# Autodesk Inventor assembly: LowerBody_MIR
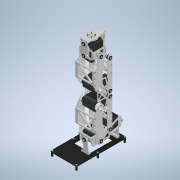
[picture p0: Inventor's stored thumbnail of the model, 180x180]
Saved by Autodesk Inventor 2020.4 (Build 244396000, 396)
## iProperties
Created: 2021-10-01
Part Number: LowerBody_MIR
Document SubType Name: Assembly
Designer: Masato
Mass: 1009.03 g
Surface Area: 2721.67 cm^2
Volume: 456.516 cm^3
Density: 2.21029 g/cm^3
Author: Masato
## Documents named in this file (14)
- C:\Users\Masato\Documents\Inventor\CIT Brains_Inventor\OpenPlatform_ver3_0\LowerBody\LowerBody_MIR.iam
- C:\Users\Masato\Documents\Inventor\CIT Brains_Inventor\OpenPlatform_ver3_0\LowerBody\Ankle\Ankle.iam
- C:\Users\Masato\Documents\Inventor\CIT Brains_Inventor\OpenPlatform_ver3_0\LowerBody\Ankle\Ankle_side_pitch.iam
- C:\Users\Masato\Documents\Inventor\CIT Brains_Inventor\OpenPlatform_ver3_0\LowerBody\Knee\Knee.iam
- C:\Users\Masato\Documents\Inventor\CIT Brains_Inventor\OpenPlatform_ver3_0\LowerBody\Leg_joit\Leg_joint_roll_pitch.iam
- C:\Users\Masato\Documents\Inventor\CIT Brains_Inventor\OpenPlatform_ver3_0\LowerBody\Leg_joit\Leg_joint_roll_yaw.iam
- C:\Users\Masato\Documents\Inventor\CIT Brains_Inventor\OpenPlatform_ver3_0\LowerBody\Slider_crank\Slider_crank_mechanism.iam
- C:\Users\Masato\Documents\Inventor\CIT Brains_Inventor\OpenPlatform_ver3_0\LowerBody\Link\BackLink.iam
- C:\Users\Masato\Documents\Inventor\CIT Brains_Inventor\OpenPlatform_ver3_0\LowerBody\Link\FrontLink.iam
- C:\Users\Masato\Documents\Inventor\CIT Brains_Inventor\OpenPlatform_ver3_0\Ready_Made\Screw\M2_6-6.ipt
- C:\Users\Masato\Documents\Inventor\CIT Brains_Inventor\OpenPlatform_ver3_0\Ready_Made\Screw\M3-6.ipt
- C:\Users\Masato\Documents\Inventor\CIT Brains_Inventor\OpenPlatform_ver3_0\Ready_Made\Screw\M2_6-10.ipt
- C:\Users\Masato\Documents\Inventor\CIT Brains_Inventor\OpenPlatform_ver3_0\Ready_Made\Screw\M3-8.ipt
- C:\Users\Masato\Documents\Inventor\CIT Brains_Inventor\OpenPlatform_ver3_0\LowerBody\Foot\Foot_MIR.iam
## Components (64 placed, 13 different names)
1. Ankle:1 [sub-assembly] — 挿入:21, 挿入:22, 挿入:67
2. Ankle_side_pitch:1 [sub-assembly] — 挿入:21, フラッシュ:5, 挿入:36, 挿入:35, 挿入:23, 挿入:24, 挿入:25, 挿入:26
3. Ankle_side_pitch:2 [sub-assembly] — フラッシュ:5, 挿入:22, 挿入:27, 挿入:28, 挿入:29, 挿入:30
4. Knee:1 [sub-assembly] — 挿入:33, 挿入:31, 挿入:34, 挿入:32
5. Leg_joint_roll_pitch:1 [sub-assembly] — 挿入:11, 挿入:2, 挿入:38, 挿入:37, 挿入:1
6. Leg_joint_roll_yaw:1 [sub-assembly] — 挿入:11, フラッシュ:4, フラッシュ:3, メイト:1, 角度:2, 挿入:12, 挿入:13, 挿入:14, 角度:8, 角度:9
7. Slider_crank_mechanism:1 [sub-assembly] — 挿入:2, 角度:1, 挿入:10, 挿入:9, 挿入:8, 挿入:7
8. BackLink:1 [sub-assembly] — 挿入:36, 挿入:33, 挿入:42, 挿入:46, 挿入:64, 挿入:66
9. FrontLink:1 [sub-assembly] — 挿入:35, 挿入:31, 挿入:51, 挿入:52, 挿入:53, 挿入:54, 挿入:59, 挿入:60, 挿入:61, 挿入:62, 挿入:63, 挿入:65, 角度:6
10. BackLink:2 [sub-assembly] — 挿入:38, 挿入:34, 挿入:39, 挿入:44, 挿入:41, 挿入:45
11. FrontLink:2 [sub-assembly] — 角度:2, 挿入:37, 挿入:32, 挿入:40, 挿入:43, 挿入:47, 挿入:48, 挿入:49, 挿入:50, 挿入:56, 挿入:57, 挿入:58, 挿入:55
12. Slider_crank_mechanism:2 [sub-assembly] — 挿入:12, 角度:1, 挿入:1, 挿入:3, 挿入:4, 挿入:5, 挿入:6
13. M2_6-6:1 — 挿入:3
14. M2_6-6:2 — 挿入:4
15. M2_6-6:3 — 挿入:5
16. M2_6-6:4 — 挿入:6
17. M2_6-6:5 — 挿入:10
18. M2_6-6:6 — 挿入:9
19. M2_6-6:7 — 挿入:8
20. M2_6-6:8 — 挿入:7
21. M3-6:1 — 挿入:13
22. M3-6:2 — 挿入:14
23. M3-6:3 — 挿入:68
24. M2_6-6:9 — 挿入:71
25. M2_6-6:10 — 挿入:69
26. M2_6-6:11 — 挿入:72
27. M2_6-6:12 — 挿入:70
28. M2_6-6:13 — 挿入:23
29. M2_6-6:14 — 挿入:24
30. M2_6-6:15 — 挿入:25
31. M2_6-6:16 — 挿入:26
32. M2_6-6:17 — 挿入:27
33. M2_6-6:18 — 挿入:28
34. M2_6-6:19 — 挿入:29
35. M2_6-6:20 — 挿入:30
36. M3-6:4 — 挿入:40
37. M3-6:5 — 挿入:39
38. M3-6:6 — 挿入:44
39. M3-6:7 — 挿入:43
40. M3-6:8 — 挿入:41
41. M3-6:9 — 挿入:45
42. M3-6:10 — 挿入:42
43. M3-6:11 — 挿入:46
44. M2_6-10:1 — 挿入:47
45. M2_6-10:2 — 挿入:48
46. M2_6-10:3 — 挿入:49
47. M2_6-10:4 — 挿入:50
48. M2_6-10:5 — 挿入:56
49. M2_6-10:6 — 挿入:57
50. M2_6-10:7 — 挿入:58
51. M2_6-10:8 — 挿入:55
52. M2_6-10:9 — 挿入:51
53. M2_6-10:10 — 挿入:52
54. M2_6-10:11 — 挿入:53
55. M2_6-10:12 — 挿入:54
56. M2_6-10:13 — 挿入:59
57. M2_6-10:14 — 挿入:60
58. M2_6-10:15 — 挿入:61
59. M2_6-10:16 — 挿入:62
60. M3-8:1 — 挿入:63
61. M3-8:2 — 挿入:64
62. M3-8:3 — 挿入:66
63. M3-8:4 — 挿入:65
64. Foot_MIR:1 [sub-assembly] — 挿入:67, 挿入:68, 挿入:69, 挿入:70, 挿入:71, 挿入:72, 角度:6, 角度:8, 角度:9
## Relationships (75: Insert 66, Angle 5, Flush 2, Mate 2)
- 挿入:21 [Insert]: Ankle:1 ↔ Ankle_side_pitch:1
- フラッシュ:5 [Flush]: Ankle_side_pitch:1 ↔ Ankle_side_pitch:2
- 挿入:22 [Insert]: Ankle:1 ↔ Ankle_side_pitch:2
- 挿入:11 [Insert]: Leg_joint_roll_pitch:1 ↔ Leg_joint_roll_yaw:1
- フラッシュ:4 [Mate]: Leg_joint_roll_yaw:1
- フラッシュ:3 [Flush]: Leg_joint_roll_yaw:1
- メイト:1 [Mate]: Leg_joint_roll_yaw:1
- 挿入:2 [Insert]: Leg_joint_roll_pitch:1 ↔ Slider_crank_mechanism:1
- 挿入:36 [Insert]: Ankle_side_pitch:1 ↔ BackLink:1
- 挿入:33 [Insert]: Knee:1 ↔ BackLink:1
- 挿入:35 [Insert]: Ankle_side_pitch:1 ↔ FrontLink:1
- 挿入:31 [Insert]: Knee:1 ↔ FrontLink:1
- 挿入:38 [Insert]: Leg_joint_roll_pitch:1 ↔ BackLink:2
- 挿入:34 [Insert]: Knee:1 ↔ BackLink:2
- 角度:2 [Angle] (0 deg): Leg_joint_roll_yaw:1 ↔ FrontLink:2
- 挿入:37 [Insert]: Leg_joint_roll_pitch:1 ↔ FrontLink:2
- 挿入:32 [Insert]: Knee:1 ↔ FrontLink:2
- 挿入:12 [Insert]: Leg_joint_roll_yaw:1 ↔ Slider_crank_mechanism:2
- 角度:1 [Angle] (180 deg): Slider_crank_mechanism:1 ↔ Slider_crank_mechanism:2
- 挿入:1 [Insert]: Leg_joint_roll_pitch:1 ↔ Slider_crank_mechanism:2
- 挿入:3 [Insert]: Slider_crank_mechanism:2 ↔ M2_6-6:1
- 挿入:4 [Insert]: Slider_crank_mechanism:2 ↔ M2_6-6:2
- 挿入:5 [Insert]: Slider_crank_mechanism:2 ↔ M2_6-6:3
- 挿入:6 [Insert]: Slider_crank_mechanism:2 ↔ M2_6-6:4
- 挿入:10 [Insert]: Slider_crank_mechanism:1 ↔ M2_6-6:5
- 挿入:9 [Insert]: Slider_crank_mechanism:1 ↔ M2_6-6:6
- 挿入:8 [Insert]: Slider_crank_mechanism:1 ↔ M2_6-6:7
- 挿入:7 [Insert]: Slider_crank_mechanism:1 ↔ M2_6-6:8
- 挿入:13 [Insert]: Leg_joint_roll_yaw:1 ↔ M3-6:1
- 挿入:14 [Insert]: Leg_joint_roll_yaw:1 ↔ M3-6:2
- 挿入:23 [Insert]: Ankle_side_pitch:1 ↔ M2_6-6:13
- 挿入:24 [Insert]: Ankle_side_pitch:1 ↔ M2_6-6:14
- 挿入:25 [Insert]: Ankle_side_pitch:1 ↔ M2_6-6:15
- 挿入:26 [Insert]: Ankle_side_pitch:1 ↔ M2_6-6:16
- 挿入:27 [Insert]: Ankle_side_pitch:2 ↔ M2_6-6:17
- 挿入:28 [Insert]: Ankle_side_pitch:2 ↔ M2_6-6:18
- 挿入:29 [Insert]: Ankle_side_pitch:2 ↔ M2_6-6:19
- 挿入:30 [Insert]: Ankle_side_pitch:2 ↔ M2_6-6:20
- 挿入:40 [Insert]: FrontLink:2 ↔ M3-6:4
- 挿入:39 [Insert]: BackLink:2 ↔ M3-6:5
- 挿入:44 [Insert]: BackLink:2 ↔ M3-6:6
- 挿入:43 [Insert]: FrontLink:2 ↔ M3-6:7
- 挿入:41 [Insert]: BackLink:2 ↔ M3-6:8
- 挿入:45 [Insert]: BackLink:2 ↔ M3-6:9
- 挿入:42 [Insert]: BackLink:1 ↔ M3-6:10
- 挿入:46 [Insert]: BackLink:1 ↔ M3-6:11
- 挿入:47 [Insert]: FrontLink:2 ↔ M2_6-10:1
- 挿入:48 [Insert]: FrontLink:2 ↔ M2_6-10:2
- 挿入:49 [Insert]: FrontLink:2 ↔ M2_6-10:3
- 挿入:50 [Insert]: FrontLink:2 ↔ M2_6-10:4
- 挿入:56 [Insert]: FrontLink:2 ↔ M2_6-10:5
- 挿入:57 [Insert]: FrontLink:2 ↔ M2_6-10:6
- 挿入:58 [Insert]: FrontLink:2 ↔ M2_6-10:7
- 挿入:55 [Insert]: FrontLink:2 ↔ M2_6-10:8
- 挿入:51 [Insert]: FrontLink:1 ↔ M2_6-10:9
- 挿入:52 [Insert]: FrontLink:1 ↔ M2_6-10:10
- 挿入:53 [Insert]: FrontLink:1 ↔ M2_6-10:11
- 挿入:54 [Insert]: FrontLink:1 ↔ M2_6-10:12
- 挿入:59 [Insert]: FrontLink:1 ↔ M2_6-10:13
- 挿入:60 [Insert]: FrontLink:1 ↔ M2_6-10:14
- 挿入:61 [Insert]: FrontLink:1 ↔ M2_6-10:15
- 挿入:62 [Insert]: FrontLink:1 ↔ M2_6-10:16
- 挿入:63 [Insert]: FrontLink:1 ↔ M3-8:1
- 挿入:64 [Insert]: BackLink:1 ↔ M3-8:2
- 挿入:66 [Insert]: BackLink:1 ↔ M3-8:3
- 挿入:65 [Insert]: FrontLink:1 ↔ M3-8:4
- 挿入:67 [Insert]: Ankle:1 ↔ Foot_MIR:1
- 挿入:68 [Insert]: M3-6:3 ↔ Foot_MIR:1
- 挿入:69 [Insert]: M2_6-6:10 ↔ Foot_MIR:1
- 挿入:70 [Insert]: M2_6-6:12 ↔ Foot_MIR:1
- 挿入:71 [Insert]: M2_6-6:9 ↔ Foot_MIR:1
- 挿入:72 [Insert]: M2_6-6:11 ↔ Foot_MIR:1
- 角度:6 [Angle] (0 deg): FrontLink:1 ↔ Foot_MIR:1
- 角度:8 [Angle] (0 deg): Leg_joint_roll_yaw:1 ↔ Foot_MIR:1
- 角度:9 [Angle] (0 deg): Leg_joint_roll_yaw:1 ↔ Foot_MIR:1
